# Autodesk Inventor assembly: HatpHexa
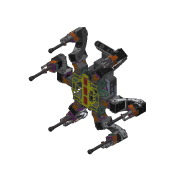
[picture p0: Inventor's stored thumbnail of the model, 180x180]
Saved by Autodesk Inventor 2019.4 (Build 234330000, 330)
## iProperties
Created: 2018-12-18
Part Number: HatpHexa
Material: 一般
Document SubType Name: Assembly
Designer: y6tada
Author: y6tada
## Documents named in this file (7)
- C:\Workspace\Yunit8-HaptHexa\Hardware\Inventor\HatpHexa.iam
- C:\Workspace\Yunit8-HaptHexa\Hardware\Inventor\Thorax\_Thorax.iam
- C:\Workspace\Yunit8-HaptHexa\Hardware\Inventor\Coxa\_Coxa.iam
- C:\Workspace\Yunit8-HaptHexa\Hardware\Inventor\Femur\_Femur.iam
- C:\Workspace\Yunit8-HaptHexa\Hardware\Inventor\Tibia\_Tibia.iam
- C:\Workspace\Yunit8-HaptHexa\Hardware\Inventor\Computer\_Computer.iam
- C:\Workspace\Yunit8-HaptHexa\Hardware\Inventor\Computer\Intel Realsense D435\D435_ipt.ipt
## Components (21 placed, 6 different names)
1. _Thorax:1 [sub-assembly] — メイト:2, 角度:1, メイト:11, メイト:12, メイト:17, メイト:18, 角度:2, 角度:3, メイト:1, メイト:34, メイト:35, メイト:36, メイト:37, メイト:38, メイト:39, 角度:5, 角度:6, 角度:7
2. _Computer:1 [sub-assembly] — フラッシュ:1, フラッシュ:2, 角度:4
3. D435_ipt:1 — フラッシュ:2, 角度:4
4. _Coxa:1 [sub-assembly] — メイト:1, 角度:1, メイト:2, メイト:44, メイト:45
5. _Femur:1 [sub-assembly] — メイト:44, メイト:45, メイト:46, メイト:47
6. _Tibia:1 [sub-assembly] — メイト:46, メイト:47, メイト:64
7. _Coxa:2 [sub-assembly] — メイト:11, メイト:12, 角度:2, メイト:48, メイト:49
8. _Femur:2 [sub-assembly] — メイト:48, メイト:49, メイト:50, メイト:51
9. _Tibia:2 [sub-assembly] — メイト:50, メイト:51, メイト:65
10. _Coxa:3 [sub-assembly] — メイト:17, メイト:18, 角度:3, メイト:52, メイト:53
11. _Femur:3 [sub-assembly] — メイト:52, メイト:53, メイト:54, メイト:55
12. _Tibia:3 [sub-assembly] — メイト:54, メイト:55, メイト:66
13. _Coxa:4 [sub-assembly] — メイト:36, メイト:39, メイト:56, メイト:57, 角度:5
14. _Femur:4 [sub-assembly] — メイト:56, メイト:57, メイト:58, メイト:59
15. _Tibia:4 [sub-assembly] — メイト:58, メイト:59, メイト:67
16. _Coxa:5 [sub-assembly] — メイト:35, メイト:37, 角度:6, メイト:60, メイト:61
17. _Femur:5 [sub-assembly] — メイト:60, メイト:61, メイト:62, メイト:63
18. _Tibia:5 [sub-assembly] — メイト:62, メイト:63, メイト:68
19. _Coxa:6 [sub-assembly] — メイト:34, メイト:38, メイト:40, メイト:41, 角度:7
20. _Femur:6 [sub-assembly] — メイト:40, メイト:41, メイト:42, メイト:43
21. _Tibia:6 [sub-assembly] — メイト:42, メイト:43, メイト:69
## Relationships (52: Mate 42, Angle 7, Flush 3)
- 角度:1 [Angle] (30 deg): _Thorax:1 ↔ _Coxa:1
- 角度:2 [Angle] (180 deg): _Thorax:1 ↔ _Coxa:2
- 角度:3 [Angle] (30 deg): _Thorax:1 ↔ _Coxa:3
- メイト:1 [Mate]: _Thorax:1 ↔ _Coxa:1
- メイト:2 [Mate]: _Thorax:1 ↔ _Coxa:1
- メイト:11 [Mate]: _Thorax:1 ↔ _Coxa:2
- メイト:12 [Mate]: _Thorax:1 ↔ _Coxa:2
- メイト:17 [Mate]: _Thorax:1 ↔ _Coxa:3
- メイト:18 [Mate]: _Thorax:1 ↔ _Coxa:3
- フラッシュ:1 [Flush]: _Computer:1
- メイト:34 [Mate]: _Thorax:1 ↔ _Coxa:6
- メイト:35 [Mate]: _Thorax:1 ↔ _Coxa:5
- メイト:36 [Mate]: _Thorax:1 ↔ _Coxa:4
- メイト:37 [Mate]: _Thorax:1 ↔ _Coxa:5
- メイト:38 [Mate]: _Thorax:1 ↔ _Coxa:6
- メイト:39 [Mate]: _Thorax:1 ↔ _Coxa:4
- フラッシュ:2 [Flush]: _Computer:1 ↔ D435_ipt:1
- 角度:4 [Angle] (-35 deg): _Computer:1 ↔ D435_ipt:1
- メイト:40 [Mate]: _Coxa:6 ↔ _Femur:6
- メイト:41 [Mate]: _Coxa:6 ↔ _Femur:6
- メイト:42 [Mate]: _Femur:6 ↔ _Tibia:6
- メイト:43 [Mate]: _Femur:6 ↔ _Tibia:6
- メイト:44 [Mate]: _Coxa:1 ↔ _Femur:1
- メイト:45 [Mate]: _Coxa:1 ↔ _Femur:1
- メイト:46 [Mate]: _Femur:1 ↔ _Tibia:1
- メイト:47 [Mate]: _Femur:1 ↔ _Tibia:1
- メイト:48 [Mate]: _Coxa:2 ↔ _Femur:2
- メイト:49 [Mate]: _Coxa:2 ↔ _Femur:2
- メイト:50 [Mate]: _Femur:2 ↔ _Tibia:2
- メイト:51 [Mate]: _Femur:2 ↔ _Tibia:2
- メイト:52 [Mate]: _Coxa:3 ↔ _Femur:3
- メイト:53 [Mate]: _Coxa:3 ↔ _Femur:3
- メイト:54 [Mate]: _Femur:3 ↔ _Tibia:3
- メイト:55 [Mate]: _Femur:3 ↔ _Tibia:3
- メイト:56 [Mate]: _Coxa:4 ↔ _Femur:4
- メイト:57 [Mate]: _Coxa:4 ↔ _Femur:4
- メイト:58 [Mate]: _Femur:4 ↔ _Tibia:4
- メイト:59 [Mate]: _Femur:4 ↔ _Tibia:4
- 角度:5 [Angle] (30 deg): _Thorax:1 ↔ _Coxa:4
- 角度:6 [Angle] (0 deg): _Thorax:1 ↔ _Coxa:5
- 角度:7 [Angle] (30 deg): _Thorax:1 ↔ _Coxa:6
- メイト:60 [Mate]: _Coxa:5 ↔ _Femur:5
- メイト:61 [Mate]: _Coxa:5 ↔ _Femur:5
- メイト:62 [Mate]: _Femur:5 ↔ _Tibia:5
- メイト:63 [Mate]: _Femur:5 ↔ _Tibia:5
- フラッシュ:3 [Flush] (-80 mm)
- メイト:64 [Mate]: _Tibia:1
- メイト:65 [Mate]: _Tibia:2
- メイト:66 [Mate]: _Tibia:3
- メイト:67 [Mate]: _Tibia:4
- メイト:68 [Mate]: _Tibia:5
- メイト:69 [Mate]: _Tibia:6
